# Autodesk Inventor assembly: assambly filament
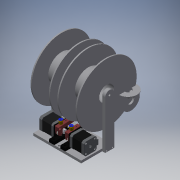
[picture p0: Inventor's stored thumbnail of the model, 180x180]
Saved by Autodesk Inventor 2016 SP1 (Build 200210100, 210)
## iProperties
Created: 2016-04-23
Part Number: assambly filament
Document SubType Name: Assembly
Designer: ubik
Author: ubik
## Documents named in this file (7)
- E:\GitHub\kossel-XXL\assambly filament.iam
- E:\GitHub\kossel-XXL\extruder assembly.iam
- E:\GitHub\kossel-XXL\extruder assembly_MIR.iam
- E:\GitHub\kossel-XXL\stl\spool main support.ipt
- E:\GitHub\kossel-XXL\spool arm support.ipt
- E:\GitHub\kossel-XXL\spool diam support.ipt
- E:\GitHub\kossel-XXL\filament spool.ipt
## Components (10 placed, 6 different names)
1. extruder assembly:3 [sub-assembly] — Flush:1, Flush:2, Mate:1, Flush:3
2. extruder assembly_MIR:1 [sub-assembly] — Flush:1, Flush:2, Mate:1
3. spool main support:1 — Flush:3, Mate:2, Flush:4, Flush:5, Flush:7, Mate:3
4. spool arm support:1 — Mate:2, Flush:4, Flush:5, Flush:6, Mate:4, Mate:5
5. spool arm support:2 — Flush:6, Flush:7, Mate:3, Mate:6, Mate:7, Mate:9
6. spool diam support:1
7. spool diam support:2
8. spool diam support:3 — Mate:6, Mate:7, Mate:8
9. filament spool:1 — Mate:8, Mate:9
10. filament spool:2 — Mate:4, Mate:5
## Relationships (16: Mate 9, Flush 7)
- Flush:1: extruder assembly:3 ↔ extruder assembly_MIR:1
- Flush:2: extruder assembly:3 ↔ extruder assembly_MIR:1
- Mate:1 (20 mm): extruder assembly:3 ↔ extruder assembly_MIR:1
- Flush:3: extruder assembly:3 ↔ spool main support:1
- Mate:2: spool main support:1 ↔ spool arm support:1
- Flush:4: spool main support:1 ↔ spool arm support:1
- Flush:5: spool main support:1 ↔ spool arm support:1
- Flush:6: spool arm support:1 ↔ spool arm support:2
- Flush:7: spool main support:1 ↔ spool arm support:2
- Mate:3: spool main support:1 ↔ spool arm support:2
- Mate:4: spool arm support:1 ↔ filament spool:2
- Mate:5: spool arm support:1 ↔ filament spool:2
- Mate:6: spool arm support:2 ↔ spool diam support:3
- Mate:7: spool arm support:2 ↔ spool diam support:3
- Mate:8: spool diam support:3 ↔ filament spool:1
- Mate:9: spool arm support:2 ↔ filament spool:1
